# Autodesk Inventor assembly: ConveyorIdleSide_20Jan
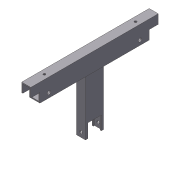
[picture p0: Inventor's stored thumbnail of the model, 180x180]
Saved by Autodesk Inventor 2012 (Build 160160000, 160)
## iProperties
Created: 2012-01-20
Part Number: ConveyorIdleSide_20Jan
Document SubType Name: Assembly
Designer: JesseK
Mass: 551.263 g
Surface Area: 1313.83 cm^2
Volume: 203.418 cm^3
Density: 2.71 g/cm^3
Author: JesseK
## Documents named in this file (3)
- Z:\UserData\Documents\Inventor\team1885frc\Robot2012\Drawings\ConveyorIdleSide_20Jan.iam
- Z:\UserData\Documents\Inventor\team1885frc\Robot2012\Conveyor2\Frame_MainHorizontalMount.ipt
- Z:\UserData\Documents\Inventor\team1885frc\Robot2012\Conveyor2\Frame_LowerRollerMount.ipt
## Components (2 placed, 2 different names)
1. Frame_MainHorizontalMount:1 — Mate:1, Flush:1, Flush:2
2. Frame_LowerRollerMount:1 — Mate:1, Flush:1, Flush:2
## Relationships (3: Flush 2, Mate 1)
- Mate:1: Frame_MainHorizontalMount:1 ↔ Frame_LowerRollerMount:1
- Flush:1: Frame_MainHorizontalMount:1 ↔ Frame_LowerRollerMount:1
- Flush:2 (152.4 mm): Frame_MainHorizontalMount:1 ↔ Frame_LowerRollerMount:1
